# Autodesk Inventor assembly: chassis_2-02
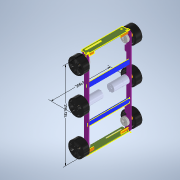
[picture p0: Inventor's stored thumbnail of the model, 180x180]
Saved by Autodesk Inventor 2022 (Build 260153000, 153)
## iProperties
Created: 2023-03-24
Part Number: chassis_2-02
Document SubType Name: Assembly
Designer: Johnny Jou
Author: Johnny Jou
## Documents named in this file (12)
- C:\Users\Johnny Jou\Documents\GitHub\Areo_Rider_Cabin\car\chassis_2.iam
- C:\Users\Johnny Jou\Documents\GitHub\Areo_Rider_Cabin\car\chassis_1_1.ipt
- C:\Users\Johnny Jou\Documents\GitHub\Areo_Rider_Cabin\car\chassis_1_2.ipt
- C:\Users\Johnny Jou\Documents\GitHub\Areo_Rider_Cabin\car\chassis_1_3.ipt
- C:\Users\Johnny Jou\Documents\GitHub\Areo_Rider_Cabin\car\chassis_1_4.ipt
- C:\Users\Johnny Jou\Documents\GitHub\Areo_Rider_Cabin\car\wheel.ipt
- C:\Users\Johnny Jou\Documents\GitHub\Areo_Rider_Cabin\car\wheel_base_cover.ipt
- C:\Users\Johnny Jou\Documents\GitHub\Areo_Rider_Cabin\car\bearing.iam
- C:\Users\Johnny Jou\Documents\GitHub\Areo_Rider_Cabin\car\axle 4_20.ipt
- C:\Users\Johnny Jou\Documents\GitHub\Areo_Rider_Cabin\car\Coupling.ipt
- C:\Users\Johnny Jou\Documents\GitHub\Areo_Rider_Cabin\motor\25GA370.ipt
- C:\Users\Johnny Jou\Documents\GitHub\Areo_Rider_Cabin\car\chassis_1_1\chassis_1_1-01.ipt
## Components (36 placed, 11 different names)
1. chassis_1_1:1 — 貼合:1, 齊平:1, 齊平:2, 貼合:3, 貼合:4, 貼合:6, 齊平:5, 貼合:7, 貼合:8, 齊平:6, 貼合:9, 齊平:8, 齊平:12, 貼合:40, 貼合:41, 貼合:42, 貼合:43, 貼合:44, 貼合:45, 貼合:66, 貼合:67, 貼合:68
2. chassis_1_2:1 — 貼合:1, 齊平:2, 齊平:3, 貼合:10, 齊平:7, 齊平:10
3. chassis_1_2:2 — 齊平:1, 齊平:3, 貼合:3, 貼合:4, 貼合:11, 齊平:13, 齊平:16, 齊平:26
4. chassis_1_3:1 — 貼合:6, 齊平:5, 貼合:7, 齊平:25
5. chassis_1_3:2 — 貼合:8, 齊平:6, 貼合:9, 貼合:78
6. chassis_1_4:1 — 貼合:10, 齊平:7, 齊平:8, 齊平:11
7. chassis_1_4:2 — 齊平:10, 齊平:11, 齊平:28
8. chassis_1_4:3 — 貼合:11, 齊平:12, 齊平:13, 齊平:14
9. chassis_1_4:4 — 齊平:14, 齊平:16, 齊平:27
10. wheel:1 — 貼合:16, 貼合:17, 貼合:18
11. wheel_base_cover:1 — 貼合:12, 齊平:17, 貼合:15, 貼合:41, 貼合:42
12. 軸承:1 [sub-assembly] — 貼合:12, 齊平:17, 貼合:13, 齊平:18
13. axle 4_20:1 — 貼合:13, 齊平:18, 貼合:14, 貼合:40
14. Coupling:1 — 貼合:14, 貼合:15, 貼合:16, 貼合:17, 貼合:18
15. wheel:2
16. wheel_base_cover:2 — 貼合:43, 貼合:44, 貼合:45
17. 軸承:2 [sub-assembly]
18. axle 4_20:2
19. Coupling:2
20. wheel:3
21. wheel_base_cover:3 — 貼合:71, 貼合:72, 貼合:77
22. 軸承:3 [sub-assembly]
23. axle 4_20:3
24. Coupling:3
25. wheel:4
26. wheel_base_cover:4 — 貼合:69, 貼合:70, 貼合:76
27. 軸承:4 [sub-assembly]
28. axle 4_20:4
29. Coupling:4
30. wheel:5
31. Coupling:5 — 貼合:59, 貼合:60
32. 25GA370:1 — 貼合:59, 貼合:60, 貼合:66, 貼合:67, 貼合:68
33. wheel:6
34. Coupling:6
35. 25GA370:2 — 貼合:73, 貼合:74, 貼合:75
36. chassis_1_1-01:2 — 貼合:69, 貼合:70, 貼合:71, 貼合:72, 貼合:73, 貼合:74, 貼合:75, 貼合:76, 貼合:77, 貼合:78, 齊平:25, 齊平:26, 齊平:27, 齊平:28
## Relationships (91: Mate 66, Flush 25)
- 貼合:1 [Mate]: chassis_1_1:1 ↔ chassis_1_2:1
- 齊平:1 [Flush]: chassis_1_1:1 ↔ chassis_1_2:2
- 齊平:2 [Flush]: chassis_1_1:1 ↔ chassis_1_2:1
- 齊平:3 [Flush]: chassis_1_2:1 ↔ chassis_1_2:2
- 貼合:3 [Mate]: chassis_1_1:1 ↔ chassis_1_2:2
- 貼合:4 [Mate]: chassis_1_1:1 ↔ chassis_1_2:2
- 貼合:6 [Mate]: chassis_1_1:1 ↔ chassis_1_3:1
- 齊平:5 [Flush]: chassis_1_1:1 ↔ chassis_1_3:1
- 貼合:7 [Mate]: chassis_1_1:1 ↔ chassis_1_3:1
- 貼合:8 [Mate]: chassis_1_1:1 ↔ chassis_1_3:2
- 齊平:6 [Flush]: chassis_1_1:1 ↔ chassis_1_3:2
- 貼合:9 [Mate]: chassis_1_1:1 ↔ chassis_1_3:2
- 貼合:10 [Mate]: chassis_1_2:1 ↔ chassis_1_4:1
- 齊平:7 [Flush]: chassis_1_2:1 ↔ chassis_1_4:1
- 齊平:8 [Flush]: chassis_1_1:1 ↔ chassis_1_4:1
- 齊平:10 [Flush]: chassis_1_2:1 ↔ chassis_1_4:2
- 齊平:11 [Flush]: chassis_1_4:1 ↔ chassis_1_4:2
- 貼合:11 [Mate]: chassis_1_2:2 ↔ chassis_1_4:3
- 齊平:12 [Flush]: chassis_1_1:1 ↔ chassis_1_4:3
- 齊平:13 [Flush]: chassis_1_2:2 ↔ chassis_1_4:3
- 齊平:14 [Flush]: chassis_1_4:3 ↔ chassis_1_4:4
- 齊平:16 [Flush]: chassis_1_2:2 ↔ chassis_1_4:4
- 貼合:12 [Mate]: wheel_base_cover:1 ↔ 軸承:1
- 齊平:17 [Flush]: wheel_base_cover:1 ↔ 軸承:1
- 貼合:13 [Mate]: 軸承:1 ↔ axle 4_20:1
- 齊平:18 [Flush]: 軸承:1 ↔ axle 4_20:1
- 貼合:14 [Mate]: axle 4_20:1 ↔ Coupling:1
- 貼合:15 [Mate] (6 mm): wheel_base_cover:1 ↔ Coupling:1
- 貼合:16 [Mate]: wheel:1 ↔ Coupling:1
- 貼合:17 [Mate]: wheel:1 ↔ Coupling:1
- 貼合:18 [Mate]: wheel:1 ↔ Coupling:1
- [Mate]: wheel_base_cover:2 ↔ 軸承:2
- [Flush]: wheel_base_cover:2 ↔ 軸承:2
- [Mate]: 軸承:2 ↔ axle 4_20:2
- [Flush]: 軸承:2 ↔ axle 4_20:2
- [Mate]: axle 4_20:2 ↔ Coupling:2
- [Mate] (6 mm): wheel_base_cover:2 ↔ Coupling:2
- [Mate]: wheel:2 ↔ Coupling:2
- [Mate]: wheel:2 ↔ Coupling:2
- [Mate]: wheel:2 ↔ Coupling:2
- [Mate]: wheel_base_cover:3 ↔ 軸承:3
- [Flush]: wheel_base_cover:3 ↔ 軸承:3
- [Mate]: 軸承:3 ↔ axle 4_20:3
- [Flush]: 軸承:3 ↔ axle 4_20:3
- [Mate]: axle 4_20:3 ↔ Coupling:3
- [Mate] (6 mm): wheel_base_cover:3 ↔ Coupling:3
- [Mate]: wheel:3 ↔ Coupling:3
- [Mate]: wheel:3 ↔ Coupling:3
- [Mate]: wheel:3 ↔ Coupling:3
- [Mate]: wheel_base_cover:4 ↔ 軸承:4
- [Flush]: wheel_base_cover:4 ↔ 軸承:4
- [Mate]: 軸承:4 ↔ axle 4_20:4
- [Flush]: 軸承:4 ↔ axle 4_20:4
- [Mate]: axle 4_20:4 ↔ Coupling:4
- [Mate] (6 mm): wheel_base_cover:4 ↔ Coupling:4
- [Mate]: wheel:4 ↔ Coupling:4
- [Mate]: wheel:4 ↔ Coupling:4
- [Mate]: wheel:4 ↔ Coupling:4
- 貼合:40 [Mate]: chassis_1_1:1 ↔ axle 4_20:1
- 貼合:41 [Mate]: chassis_1_1:1 ↔ wheel_base_cover:1
- 貼合:42 [Mate]: chassis_1_1:1 ↔ wheel_base_cover:1
- 貼合:43 [Mate]: chassis_1_1:1 ↔ wheel_base_cover:2
- 貼合:44 [Mate]: chassis_1_1:1 ↔ wheel_base_cover:2
- 貼合:45 [Mate]: chassis_1_1:1 ↔ wheel_base_cover:2
- [Mate]: wheel:5 ↔ Coupling:5
- [Mate]: wheel:5 ↔ Coupling:5
- [Mate]: wheel:5 ↔ Coupling:5
- 貼合:59 [Mate]: Coupling:5 ↔ 25GA370:1
- 貼合:60 [Mate] (6 mm): Coupling:5 ↔ 25GA370:1
- [Mate]: wheel:6 ↔ Coupling:6
- [Mate]: wheel:6 ↔ Coupling:6
- [Mate]: wheel:6 ↔ Coupling:6
- [Mate]: Coupling:6 ↔ 25GA370:2
- [Mate] (6 mm): Coupling:6 ↔ 25GA370:2
- 貼合:66 [Mate]: chassis_1_1:1 ↔ 25GA370:1
- 貼合:67 [Mate]: chassis_1_1:1 ↔ 25GA370:1
- 貼合:68 [Mate]: chassis_1_1:1 ↔ 25GA370:1
- 貼合:69 [Mate]: wheel_base_cover:4 ↔ chassis_1_1-01:2
- 貼合:70 [Mate]: wheel_base_cover:4 ↔ chassis_1_1-01:2
- 貼合:71 [Mate]: wheel_base_cover:3 ↔ chassis_1_1-01:2
- 貼合:72 [Mate]: wheel_base_cover:3 ↔ chassis_1_1-01:2
- 貼合:73 [Mate]: 25GA370:2 ↔ chassis_1_1-01:2
- 貼合:74 [Mate]: 25GA370:2 ↔ chassis_1_1-01:2
- 貼合:75 [Mate]: 25GA370:2 ↔ chassis_1_1-01:2
- 貼合:76 [Mate]: wheel_base_cover:4 ↔ chassis_1_1-01:2
- 貼合:77 [Mate]: wheel_base_cover:3 ↔ chassis_1_1-01:2
- 貼合:78 [Mate]: chassis_1_3:2 ↔ chassis_1_1-01:2
- 齊平:25 [Flush]: chassis_1_3:1 ↔ chassis_1_1-01:2
- 齊平:26 [Flush]: chassis_1_2:2 ↔ chassis_1_1-01:2
- 齊平:27 [Flush]: chassis_1_4:4 ↔ chassis_1_1-01:2
- 齊平:28 [Flush]: chassis_1_4:2 ↔ chassis_1_1-01:2
## Named parameters: d118_d109 = 0 mm, d119_d110 = 0 mm, d120_d111 = 0 mm, d121_d112 = 0 mm, d122_d113 = 0 mm, d123_d114 = 6 mm, d124_d115 = 0 mm, d125_d116 = 0 mm, d126_d117 = 0 mm, d127_d109 = 0 mm, d128_d110 = 0 mm, d129_d111 = 0 mm, d130_d112 = 0 mm, d131_d113 = 0 mm, d132_d114 = 6 mm, d133_d115 = 0 mm, d134_d116 = 0 mm, d135_d117 = 0 mm, d136_d109 = 0 mm, d137_d110 = 0 mm, d138_d111 = 0 mm, d139_d112 = 0 mm, d140_d113 = 0 mm, d141_d114 = 6 mm, d142_d115 = 0 mm, d143_d116 = 0 mm, d144_d117 = 0 mm, d163_d115 = 0 mm, d164_d116 = 0 mm, d165_d117 = 0 mm, d168_d163_d115 = 0 mm, d169_d164_d116 = 0 mm, d170_d165_d117 = 0 mm, d171_d166 = 0 mm, d172_d167 = 6 mm
